# Autodesk Inventor assembly: Hinge Assembly
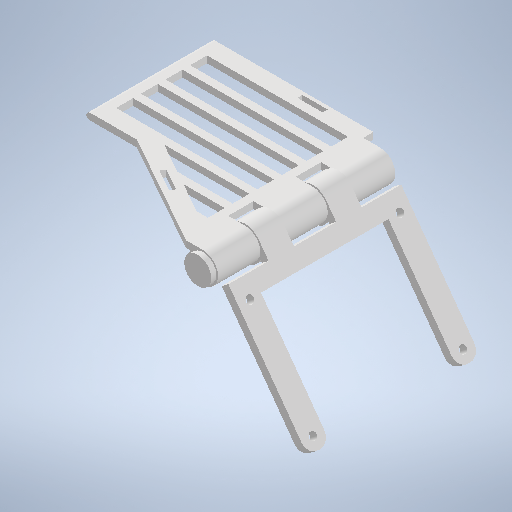
[picture p0: Inventor's stored thumbnail of the model, 512x512]
Saved by Autodesk Inventor 2025.1 (Build 291241020, 241B)
## iProperties
Created: 2024-10-26
Part Number: Hinge Assembly
Document SubType Name: Assembly
Designer: nitve
Mass: 62.073 g
Surface Area: 376.618 cm^2
Volume: 62.073 cm^3
Density: 1 g/cm^3
Author: nitve
## Documents named in this file (4)
- C:\Users\aly_g\Downloads\School\Eng Design\P1\CAD Model\Hinge Assembly.iam
- C:\Users\aly_g\Downloads\School\Eng Design\P1\CAD Model\Hinge Part 2.ipt
- C:\Users\aly_g\Downloads\School\Eng Design\P1\CAD Model\Hinge.ipt
- C:\Users\aly_g\Downloads\School\Eng Design\P1\CAD Model\pin.ipt
## Components (3 placed, 3 different names)
1. Hinge Part 2:1 — Insert:1, Insert:2
2. Hinge:1 — Insert:2
3. pin:1 — Insert:1
## Relationships (2: Insert 2)
- Insert:1: Hinge Part 2:1 ↔ pin:1
- Insert:2: Hinge Part 2:1 ↔ Hinge:1
